# Autodesk Inventor assembly: Raspberry Pi Pico-R3
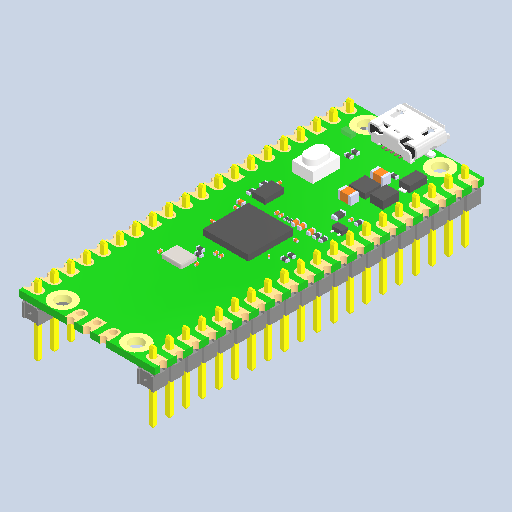
[picture p0: Inventor's stored thumbnail of the model, 512x512]
Saved by Autodesk Inventor 2023 (Build 270158000, 158)
## iProperties
Created: 2021-01-27
Part Number: Raspberry Pi Pico-R3
Document SubType Name: Assembly
Designer: graeme
Sending System: SolidWorks 2018
Last Author: NUC
Last Saved: 2021-02-07
Author: graeme
## Documents named in this file (46)
- C:\Work\Projects\swc_perturbation_treadmill\mCAD\Neural Link Box\raspberry-pi-pico\Raspberry Pi Pico-R3.iam
- C:\Work\Projects\swc_perturbation_treadmill\mCAD\Neural Link Box\raspberry-pi-pico\PCB, Raspberry Pi Pico-R3.ipt
- C:\Work\Projects\swc_perturbation_treadmill\mCAD\Neural Link Box\raspberry-pi-pico\MicroUSB Port, Raspberry Pi Pico-R3.ipt
- C:\Work\Projects\swc_perturbation_treadmill\mCAD\Neural Link Box\raspberry-pi-pico\RP2040 Microcontroller, Raspberry Pi Pico-R3.ipt
- C:\Work\Projects\swc_perturbation_treadmill\mCAD\Neural Link Box\raspberry-pi-pico\SW1, Tact Switch, Raspberry Pi Pico-R3.ipt
- C:\Work\Projects\swc_perturbation_treadmill\mCAD\Neural Link Box\raspberry-pi-pico\D1, Diode, Schottky, Raspberry Pi Pico-R3.ipt
- C:\Work\Projects\swc_perturbation_treadmill\mCAD\Neural Link Box\raspberry-pi-pico\D2, QSME-C194, LED, Raspberry Pi Pico-R3.ipt
- C:\Work\Projects\swc_perturbation_treadmill\mCAD\Neural Link Box\raspberry-pi-pico\L1, Inductor, Raspberry Pi Pico-R3.ipt
- C:\Work\Projects\swc_perturbation_treadmill\mCAD\Neural Link Box\raspberry-pi-pico\U2, RT6150B-33GQW, Buck Boost Converter, Raspberry Pi Pico-R3.ipt
- C:\Work\Projects\swc_perturbation_treadmill\mCAD\Neural Link Box\raspberry-pi-pico\U3, W25Q16JVUXIQ, Serial NOR Flash 16 Mbit, Raspberry Pi Pico-R3.ipt
- C:\Work\Projects\swc_perturbation_treadmill\mCAD\Neural Link Box\raspberry-pi-pico\Q1, MOSFET, DMG1012T, Raspberry Pi Pico-R3.ipt
- C:\Work\Projects\swc_perturbation_treadmill\mCAD\Neural Link Box\raspberry-pi-pico\X1, X12M000000S096, 12 Mhz Crystal Resonator, Raspberry Pi Pico-R3.ipt
- C:\Work\Projects\swc_perturbation_treadmill\mCAD\Neural Link Box\raspberry-pi-pico\SMD Resistor, Configurable, Raspberry Pi Pico-R3.ipt
- C:\Work\Projects\swc_perturbation_treadmill\mCAD\Neural Link Box\raspberry-pi-pico\SMD Resistor, Configurable, Raspberry Pi Pico-R3_R2.ipt
- C:\Work\Projects\swc_perturbation_treadmill\mCAD\Neural Link Box\raspberry-pi-pico\SMD Resistor, Configurable, Raspberry Pi Pico-R3_R3.ipt
- C:\Work\Projects\swc_perturbation_treadmill\mCAD\Neural Link Box\raspberry-pi-pico\SMD Resistor, Configurable, Raspberry Pi Pico-R3_R4.ipt
- C:\Work\Projects\swc_perturbation_treadmill\mCAD\Neural Link Box\raspberry-pi-pico\SMD Resistor, Configurable, Raspberry Pi Pico-R3_R5.ipt
- C:\Work\Projects\swc_perturbation_treadmill\mCAD\Neural Link Box\raspberry-pi-pico\SMD Resistor, Configurable, Raspberry Pi Pico-R3_R6.ipt
- C:\Work\Projects\swc_perturbation_treadmill\mCAD\Neural Link Box\raspberry-pi-pico\SMD Resistor, Configurable, Raspberry Pi Pico-R3_R7.ipt
- C:\Work\Projects\swc_perturbation_treadmill\mCAD\Neural Link Box\raspberry-pi-pico\SMD Resistor, Configurable, Raspberry Pi Pico-R3_R8.ipt
- C:\Work\Projects\swc_perturbation_treadmill\mCAD\Neural Link Box\raspberry-pi-pico\SMD Resistor, Configurable, Raspberry Pi Pico-R3_R9.ipt
- C:\Work\Projects\swc_perturbation_treadmill\mCAD\Neural Link Box\raspberry-pi-pico\SMD Resistor, Configurable, Raspberry Pi Pico-R3_R10.ipt
- C:\Work\Projects\swc_perturbation_treadmill\mCAD\Neural Link Box\raspberry-pi-pico\SMD Resistor, Configurable, Raspberry Pi Pico-R3_R11.ipt
- C:\Work\Projects\swc_perturbation_treadmill\mCAD\Neural Link Box\raspberry-pi-pico\SMD Resistor, Configurable, Raspberry Pi Pico-R3_R12.ipt
- C:\Work\Projects\swc_perturbation_treadmill\mCAD\Neural Link Box\raspberry-pi-pico\SMD Resistor, Configurable, Raspberry Pi Pico-R3_R13.ipt
- C:\Work\Projects\swc_perturbation_treadmill\mCAD\Neural Link Box\raspberry-pi-pico\SMD Resistor, Configurable, Raspberry Pi Pico-R3_R14.ipt
- C:\Work\Projects\swc_perturbation_treadmill\mCAD\Neural Link Box\raspberry-pi-pico\SMD Resistor, Configurable, Raspberry Pi Pico-R3_R15.ipt
- C:\Work\Projects\swc_perturbation_treadmill\mCAD\Neural Link Box\raspberry-pi-pico\SMD Capacitor, Configurable, Raspberry Pi Pico-R3.ipt
- C:\Work\Projects\swc_perturbation_treadmill\mCAD\Neural Link Box\raspberry-pi-pico\SMD Capacitor, Configurable, Raspberry Pi Pico-R3_C2.ipt
- C:\Work\Projects\swc_perturbation_treadmill\mCAD\Neural Link Box\raspberry-pi-pico\SMD Capacitor, Configurable, Raspberry Pi Pico-R3_C3.ipt
- C:\Work\Projects\swc_perturbation_treadmill\mCAD\Neural Link Box\raspberry-pi-pico\SMD Capacitor, Configurable, Raspberry Pi Pico-R3_C4.ipt
- C:\Work\Projects\swc_perturbation_treadmill\mCAD\Neural Link Box\raspberry-pi-pico\SMD Capacitor, Configurable, Raspberry Pi Pico-R3_C5.ipt
- C:\Work\Projects\swc_perturbation_treadmill\mCAD\Neural Link Box\raspberry-pi-pico\SMD Capacitor, Configurable, Raspberry Pi Pico-R3_C6.ipt
- C:\Work\Projects\swc_perturbation_treadmill\mCAD\Neural Link Box\raspberry-pi-pico\SMD Capacitor, Configurable, Raspberry Pi Pico-R3_C7.ipt
- C:\Work\Projects\swc_perturbation_treadmill\mCAD\Neural Link Box\raspberry-pi-pico\SMD Capacitor, Configurable, Raspberry Pi Pico-R3_C8.ipt
- C:\Work\Projects\swc_perturbation_treadmill\mCAD\Neural Link Box\raspberry-pi-pico\SMD Capacitor, Configurable, Raspberry Pi Pico-R3_C9.ipt
- C:\Work\Projects\swc_perturbation_treadmill\mCAD\Neural Link Box\raspberry-pi-pico\SMD Capacitor, Configurable, Raspberry Pi Pico-R3_C10.ipt
- C:\Work\Projects\swc_perturbation_treadmill\mCAD\Neural Link Box\raspberry-pi-pico\SMD Capacitor, Configurable, Raspberry Pi Pico-R3_C11.ipt
- C:\Work\Projects\swc_perturbation_treadmill\mCAD\Neural Link Box\raspberry-pi-pico\SMD Capacitor, Configurable, Raspberry Pi Pico-R3_C12.ipt
- C:\Work\Projects\swc_perturbation_treadmill\mCAD\Neural Link Box\raspberry-pi-pico\SMD Capacitor, Configurable, Raspberry Pi Pico-R3_C13.ipt
- C:\Work\Projects\swc_perturbation_treadmill\mCAD\Neural Link Box\raspberry-pi-pico\SMD Capacitor, Configurable, Raspberry Pi Pico-R3_C14.ipt
- C:\Work\Projects\swc_perturbation_treadmill\mCAD\Neural Link Box\raspberry-pi-pico\SMD Capacitor, Configurable, Raspberry Pi Pico-R3_C15.ipt
- C:\Work\Projects\swc_perturbation_treadmill\mCAD\Neural Link Box\raspberry-pi-pico\SMD Capacitor, Configurable, Raspberry Pi Pico-R3_C16.ipt
- C:\Work\Projects\swc_perturbation_treadmill\mCAD\Neural Link Box\raspberry-pi-pico\SMD Capacitor, Configurable, Raspberry Pi Pico-R3_C17.ipt
- C:\Work\Projects\swc_perturbation_treadmill\mCAD\Neural Link Box\raspberry-pi-pico\SMD Capacitor, Configurable, Raspberry Pi Pico-R3_C18.ipt
- C:\Work\Projects\swc_perturbation_treadmill\mCAD\Neural Link Box\raspberry-pi-pico\TSW-120-07-L-S.iam
## Components (46 placed, 14 different names)
1. PCB, Raspberry Pi Pico-R3:1 — Mate:1, Mate:2, Flush:1, Flush:2, Flush:4
2. MicroUSB Port, Raspberry Pi Pico-R3:1
3. RP2040 Microcontroller, Raspberry Pi Pico-R3:1
4. SW1, Tact Switch, Raspberry Pi Pico-R3:1
5. D1, Diode, Schottky, Raspberry Pi Pico-R3:1
6. D2, QSME-C194, LED, Raspberry Pi Pico-R3:1
7. L1, Inductor, Raspberry Pi Pico-R3:1
8. U2, RT6150B-33GQW, Buck Boost Converter, Raspberry Pi Pico-R3:1
9. U3, W25Q16JVUXIQ, Serial NOR Flash 16 Mbit, Raspberry Pi Pico-R3:1
10. Q1, MOSFET, DMG1012T, Raspberry Pi Pico-R3:1
11. X1, X12M000000S096, 12 Mhz Crystal Resonator, Raspberry Pi Pico-R3:1
12. SMD Resistor, Configurable, Raspberry Pi Pico-R3:1
13. SMD Resistor, Configurable, Raspberry Pi Pico-R3:2
14. SMD Resistor, Configurable, Raspberry Pi Pico-R3:3
15. SMD Resistor, Configurable, Raspberry Pi Pico-R3:4
16. SMD Resistor, Configurable, Raspberry Pi Pico-R3:5
17. SMD Resistor, Configurable, Raspberry Pi Pico-R3:6
18. SMD Resistor, Configurable, Raspberry Pi Pico-R3:7
19. SMD Resistor, Configurable, Raspberry Pi Pico-R3:8
20. SMD Resistor, Configurable, Raspberry Pi Pico-R3:9
21. SMD Resistor, Configurable, Raspberry Pi Pico-R3:10
22. SMD Resistor, Configurable, Raspberry Pi Pico-R3:11
23. SMD Resistor, Configurable, Raspberry Pi Pico-R3:12
24. SMD Resistor, Configurable, Raspberry Pi Pico-R3:13
25. SMD Resistor, Configurable, Raspberry Pi Pico-R3:14
26. SMD Resistor, Configurable, Raspberry Pi Pico-R3:15
27. SMD Capacitor, Configurable, Raspberry Pi Pico-R3:1
28. SMD Capacitor, Configurable, Raspberry Pi Pico-R3:2
29. SMD Capacitor, Configurable, Raspberry Pi Pico-R3:3
30. SMD Capacitor, Configurable, Raspberry Pi Pico-R3:4
31. SMD Capacitor, Configurable, Raspberry Pi Pico-R3:5
32. SMD Capacitor, Configurable, Raspberry Pi Pico-R3:6
33. SMD Capacitor, Configurable, Raspberry Pi Pico-R3:7
34. SMD Capacitor, Configurable, Raspberry Pi Pico-R3:8
35. SMD Capacitor, Configurable, Raspberry Pi Pico-R3:9
36. SMD Capacitor, Configurable, Raspberry Pi Pico-R3:10
37. SMD Capacitor, Configurable, Raspberry Pi Pico-R3:11
38. SMD Capacitor, Configurable, Raspberry Pi Pico-R3:19
39. SMD Capacitor, Configurable, Raspberry Pi Pico-R3:20
40. SMD Capacitor, Configurable, Raspberry Pi Pico-R3:21
41. SMD Capacitor, Configurable, Raspberry Pi Pico-R3:22
42. SMD Capacitor, Configurable, Raspberry Pi Pico-R3:23
43. SMD Capacitor, Configurable, Raspberry Pi Pico-R3:24
44. SMD Capacitor, Configurable, Raspberry Pi Pico-R3:18
45. TSW-120-07-L-S:1 [sub-assembly] — Mate:1, Flush:3, Flush:4
46. TSW-120-07-L-S:2 [sub-assembly] — Mate:2, Flush:1, Flush:2, Flush:3
## Relationships (6: Flush 4, Mate 2)
- Mate:1: PCB, Raspberry Pi Pico-R3:1 ↔ TSW-120-07-L-S:1
- Mate:2: PCB, Raspberry Pi Pico-R3:1 ↔ TSW-120-07-L-S:2
- Flush:1 (0.325 mm): PCB, Raspberry Pi Pico-R3:1 ↔ TSW-120-07-L-S:2
- Flush:2 (0.1 mm): PCB, Raspberry Pi Pico-R3:1 ↔ TSW-120-07-L-S:2
- Flush:3: TSW-120-07-L-S:1 ↔ TSW-120-07-L-S:2
- Flush:4 (0.325 mm): PCB, Raspberry Pi Pico-R3:1 ↔ TSW-120-07-L-S:1
